# Autodesk Inventor assembly: HbIndexFinger01
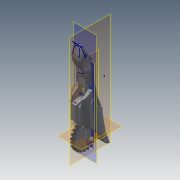
[picture p0: Inventor's stored thumbnail of the model, 180x180]
Saved by Autodesk Inventor 2015 SP1 (Build 190203100, 203)
## iProperties
Created: 2015-04-11
Part Number: HbIndexFinger01
Document SubType Name: Assembly
Designer: Yamaura
Author: Yamaura
## Documents named in this file (12)
- C:\Users\Yamaura\Documents\GitHub\HACKberry\HACKberry-hardware\3D\Inventor\Parts\HbIndexFinger01.iam
- C:\Users\Yamaura\Documents\GitHub\HACKberry\HACKberry-hardware\3D\Inventor\Parts\HbIndexInputLink02.ipt
- C:\Users\Yamaura\Documents\GitHub\HACKberry\HACKberry-hardware\3D\Inventor\Parts\TOS 0.5-6-270-5.ipt
- C:\Users\Yamaura\Documents\GitHub\HACKberry\HACKberry-hardware\3D\Inventor\Parts\HbReleaseLever01.ipt
- C:\Users\Yamaura\Documents\GitHub\HACKberry\HACKberry-hardware\3D\Inventor\Parts\HbIndexCouplerLink02.ipt
- C:\Users\Yamaura\Documents\GitHub\HACKberry\HACKberry-hardware\3D\Inventor\Parts\HbIndexCouplerLinkCover02.ipt
- C:\Users\Yamaura\Documents\GitHub\HACKberry\HACKberry-hardware\3D\Inventor\Parts\HbIndexProximalPhalanxCover02.ipt
- C:\Users\Yamaura\Documents\GitHub\HACKberry\HACKberry-hardware\3D\Inventor\Parts\HbReleaseLever02.ipt
- C:\Users\Yamaura\Documents\GitHub\HACKberry\HACKberry-hardware\3D\Inventor\Parts\HbIndexProximalPhalanx03.ipt
- C:\Users\Yamaura\Documents\GitHub\HACKberry\HACKberry-hardware\3D\Inventor\Parts\HbIndexMiddle-DistalPhalanx02.ipt
- C:\Users\Yamaura\Documents\GitHub\HACKberry\HACKberry-hardware\3D\Inventor\Parts\ScrewM2L10.ipt
- C:\Users\Yamaura\Documents\GitHub\HACKberry\HACKberry-hardware\3D\Inventor\Parts\HbIndexPosture01.ipt
## Components (16 placed, 13 different names)
1. HbIndexPosture01:1 — フラッシュ:1, フラッシュ:2, フラッシュ:3, メイト:9, メイト:11, メイト:12
2. HbIndexInputLink02_1 — メイト:9, メイト:10
3. TOS 0.5-6-270-5_1
4. TOS 0.5-6-270-5_2
5. HbReleaseLever01_1
6. HbReleaseLever01_2
7. HbIndexCouplerLink02_1
8. HbIndexCouplerLinkCover02_1 — メイト:5, メイト:6, メイト:7, メイト:8
9. HbIndexProximalPhalanxCover02_1
10. HbReleaseLever02_1
11. HbIndexProximalPhalanx03_1 — メイト:1, メイト:2, メイト:3, メイト:4
12. HbIndexMiddle-DistalPhalanx02_1 — メイト:11, メイト:12, メイト:13
13. ScrewM2L10:1 — メイト:5, メイト:6
14. ScrewM2L10:2 — メイト:7, メイト:8
15. ScrewM2L10:3 — メイト:3, メイト:4
16. ScrewM2L10:4 — メイト:1, メイト:2
## Relationships (16: Mate 13, Flush 3)
- メイト:1 [Mate]: HbIndexProximalPhalanx03_1 ↔ ScrewM2L10:4
- メイト:2 [Mate]: HbIndexProximalPhalanx03_1 ↔ ScrewM2L10:4
- メイト:3 [Mate]: HbIndexProximalPhalanx03_1 ↔ ScrewM2L10:3
- メイト:4 [Mate]: HbIndexProximalPhalanx03_1 ↔ ScrewM2L10:3
- メイト:5 [Mate]: HbIndexCouplerLinkCover02_1 ↔ ScrewM2L10:1
- メイト:6 [Mate]: HbIndexCouplerLinkCover02_1 ↔ ScrewM2L10:1
- メイト:7 [Mate]: HbIndexCouplerLinkCover02_1 ↔ ScrewM2L10:2
- メイト:8 [Mate]: HbIndexCouplerLinkCover02_1 ↔ ScrewM2L10:2
- フラッシュ:1 [Flush]: HbIndexPosture01:1
- フラッシュ:2 [Flush]: HbIndexPosture01:1
- フラッシュ:3 [Flush]: HbIndexPosture01:1
- メイト:9 [Mate]: HbIndexPosture01:1 ↔ HbIndexInputLink02_1
- メイト:10 [Mate] (-1.5 mm): HbIndexInputLink02_1
- メイト:11 [Mate]: HbIndexPosture01:1 ↔ HbIndexMiddle-DistalPhalanx02_1
- メイト:12 [Mate]: HbIndexPosture01:1 ↔ HbIndexMiddle-DistalPhalanx02_1
- メイト:13 [Mate] (-3.45 mm): HbIndexMiddle-DistalPhalanx02_1
